# Autodesk Inventor assembly: Full-Assembly
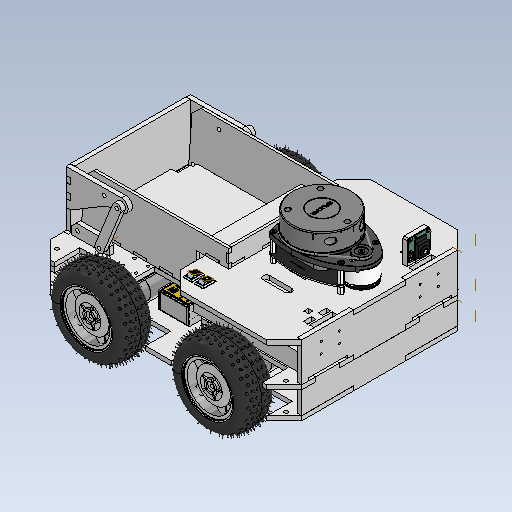
[picture p0: Inventor's stored thumbnail of the model, 512x512]
Saved by Autodesk Inventor 2025 (Build 290162000, 162)
## iProperties
Created: 2025-08-20
Part Number: Full-Assembly
Document SubType Name: Assembly
Designer: HP
Author: HP
## Documents named in this file (20)
- C:\Users\HP\Documents\GitHub\robotics-dojo-2025\CAD\Full-Assembly.iam
- C:\Users\HP\Documents\GitHub\robotics-dojo-2025\CAD\RP-lidar-A1\RP-lidar-A1.iam
- C:\Users\HP\Documents\GitHub\robotics-dojo-2025\CAD\lipo\TATTU 1800 3S.iam
- C:\Users\HP\Documents\GitHub\robotics-dojo-2025\CAD\wheel-assembly.iam
- C:\Users\HP\Documents\GitHub\robotics-dojo-2025\CAD\mainBoard.ipt
- C:\Users\HP\Documents\GitHub\robotics-dojo-2025\CAD\servo\MG-996R.ipt
- C:\Users\HP\Documents\GitHub\robotics-dojo-2025\CAD\pi\pi-assembly.iam
- C:\Users\HP\Documents\GitHub\robotics-dojo-2025\CAD\cam\raspicam_ai_assy.iam
- C:\Users\HP\Documents\GitHub\robotics-dojo-2025\CAD\frame.iam
- C:\Users\HP\Documents\GitHub\robotics-dojo-2025\CAD\servo-arm.ipt
- C:\Users\HP\Documents\GitHub\robotics-dojo-2025\CAD\lower-tipper-link.ipt
- C:\Users\HP\Documents\GitHub\robotics-dojo-2025\CAD\upper-tipper-link.ipt
- C:\Users\HP\Documents\GitHub\robotics-dojo-2025\CAD\gate.ipt
- C:\Users\HP\Documents\GitHub\robotics-dojo-2025\CAD\gate-anchor-link.ipt
- C:\Users\HP\Documents\GitHub\robotics-dojo-2025\CAD\gate-upper-link.ipt
- C:\Users\HP\Documents\GitHub\robotics-dojo-2025\CAD\power-bank.ipt
- C:\Users\HP\Documents\GitHub\robotics-dojo-2025\CAD\power-bank-bump.ipt
- C:\Users\HP\Documents\GitHub\robotics-dojo-2025\CAD\wheel\Off Road Tyre v3.ipt
- C:\Users\HP\Documents\GitHub\robotics-dojo-2025\CAD\bed_acrylic_assembly.iam
- C:\Users\HP\Documents\GitHub\robotics-dojo-2025\CAD\switch\power button.iam
## Components (29 placed, 19 different names)
1. RP-lidar-A1:1 [sub-assembly] — Insert:9, Insert:10
2. TATTU 1800 3S:1 [sub-assembly] — Mate:12, Flush:2, Mate:15
3. TATTU 1800 3S:2 [sub-assembly] — Mate:13, Flush:2, Mate:14, Mate:15, Mate:16
4. wheel-assembly:1 [sub-assembly] — Mate:4, Insert:3, Insert:4, Mate:57, Mate:58
5. wheel-assembly:2 [sub-assembly] — Mate:3, Insert:5, Insert:6, Mate:55, Mate:56
6. wheel-assembly:3 [sub-assembly] — Mate:1, Insert:1, Insert:2, Mate:16, Mate:51, Mate:52
7. wheel-assembly:4 [sub-assembly] — Mate:2, Insert:7, Insert:8, Mate:53, Mate:54
8. mainBoard:1 — Mate:5, Flush:7, Mate:23
9. MG-996R:1 — Mate:22, Insert:15, Flush:4, Flush:9
10. pi-assembly:1 [sub-assembly] — Mate:7, Flush:5, Flush:7, Mate:23, Mate:25
11. raspicam_ai_assy:1 [sub-assembly] — Mate:70, Mate:71, Mate:72
12. frame:1 [sub-assembly] — Mate:1, Mate:2, Mate:3, Mate:4, Insert:1, Insert:2, Insert:3, Insert:4, Insert:5, Insert:6, Insert:7, Insert:8, Mate:5, Mate:7, Mate:12, Mate:13, Mate:14, Insert:9, Insert:10, Mate:22, Flush:4, Flush:5, Mate:25, Flush:9, Insert:25, Insert:27, Mate:49, Mate:59, Mate:60, Flush:11, Mate:70, Mate:71, Mate:72, Mate:73, Mate:74, Mate:75, Mate:76, Mate:77, Mate:78, Angle:4
13. servo-arm:1 — Angle:1, Insert:15, Insert:18
14. lower-tipper-link:1 — Angle:1, Insert:18, Insert:19
15. upper-tipper-link:1 — Insert:19, Mate:61
16. gate:1 — Mate:38, Mate:39, Mate:40, Mate:42, Mate:43
17. gate-anchor-link:1 — Insert:25, Mate:44
18. gate-upper-link:1 — Mate:38, Mate:39, Mate:40, Mate:44, Mate:62
19. gate-upper-link:2 — Mate:42, Mate:43, Mate:46
20. gate-anchor-link:2 — Insert:27, Mate:46
21. power-bank:1 — Mate:49, Mate:50, Flush:10, Mate:59
22. power-bank-bump:1 — Mate:50, Flush:10
23. Off Road Tyre v3:1 — Mate:57, Mate:58, Angle:5
24. Off Road Tyre v3:2 — Mate:55, Mate:56, Angle:6
25. Off Road Tyre v3:3 — Mate:53, Mate:54, Angle:7
26. Off Road Tyre v3:4 — Mate:51, Mate:52, Angle:8
27. bed_acrylic_assembly:1 [sub-assembly] — Mate:60, Mate:61, Mate:62, Flush:11, Angle:4
28. power button:1 [sub-assembly] — Mate:74, Mate:75, Mate:78
29. power button:2 [sub-assembly] — Mate:73, Mate:76, Mate:77
## Relationships (72: Mate 44, Insert 15, Flush 7, Angle 6)
- Mate:1: wheel-assembly:3 ↔ frame:1
- Mate:2: wheel-assembly:4 ↔ frame:1
- Mate:3: wheel-assembly:2 ↔ frame:1
- Mate:4: wheel-assembly:1 ↔ frame:1
- Insert:1: wheel-assembly:3 ↔ frame:1
- Insert:2: wheel-assembly:3 ↔ frame:1
- Insert:3: wheel-assembly:1 ↔ frame:1
- Insert:4: wheel-assembly:1 ↔ frame:1
- Insert:5: wheel-assembly:2 ↔ frame:1
- Insert:6: wheel-assembly:2 ↔ frame:1
- Insert:7: wheel-assembly:4 ↔ frame:1
- Insert:8: wheel-assembly:4 ↔ frame:1
- Mate:5: mainBoard:1 ↔ frame:1
- Mate:7: pi-assembly:1 ↔ frame:1
- Mate:12: TATTU 1800 3S:1 ↔ frame:1
- Mate:13: TATTU 1800 3S:2 ↔ frame:1
- Flush:2: TATTU 1800 3S:1 ↔ TATTU 1800 3S:2
- Mate:14: TATTU 1800 3S:2 ↔ frame:1
- Insert:9: RP-lidar-A1:1 ↔ frame:1
- Insert:10: RP-lidar-A1:1 ↔ frame:1
- Mate:15 (15 mm): TATTU 1800 3S:1 ↔ TATTU 1800 3S:2
- Mate:16 (30 mm): TATTU 1800 3S:2 ↔ wheel-assembly:3
- Mate:22: MG-996R:1 ↔ frame:1
- Angle:1 (0 deg): servo-arm:1 ↔ lower-tipper-link:1
- Insert:15 (-4 mm): MG-996R:1 ↔ servo-arm:1
- Insert:18: servo-arm:1 ↔ lower-tipper-link:1
- Insert:19: lower-tipper-link:1 ↔ upper-tipper-link:1
- Flush:4: MG-996R:1 ↔ frame:1
- Flush:5: pi-assembly:1 ↔ frame:1
- Flush:7: mainBoard:1 ↔ pi-assembly:1
- Mate:23: mainBoard:1 ↔ pi-assembly:1
- Mate:25: pi-assembly:1 ↔ frame:1
- Flush:9: MG-996R:1 ↔ frame:1
- Insert:25: frame:1 ↔ gate-anchor-link:1
- Mate:38: gate:1 ↔ gate-upper-link:1
- Mate:39: gate:1 ↔ gate-upper-link:1
- Mate:40: gate:1 ↔ gate-upper-link:1
- Mate:42: gate:1 ↔ gate-upper-link:2
- Mate:43: gate:1 ↔ gate-upper-link:2
- Mate:44: gate-anchor-link:1 ↔ gate-upper-link:1
- Insert:27: frame:1 ↔ gate-anchor-link:2
- Mate:46: gate-upper-link:2 ↔ gate-anchor-link:2
- Mate:49: frame:1 ↔ power-bank:1
- Mate:50: power-bank:1 ↔ power-bank-bump:1
- Mate:51: wheel-assembly:3 ↔ Off Road Tyre v3:4
- Mate:52: wheel-assembly:3 ↔ Off Road Tyre v3:4
- Mate:53: wheel-assembly:4 ↔ Off Road Tyre v3:3
- Mate:54: wheel-assembly:4 ↔ Off Road Tyre v3:3
- Mate:55: wheel-assembly:2 ↔ Off Road Tyre v3:2
- Mate:56: wheel-assembly:2 ↔ Off Road Tyre v3:2
- Mate:57: wheel-assembly:1 ↔ Off Road Tyre v3:1
- Mate:58: wheel-assembly:1 ↔ Off Road Tyre v3:1
- Flush:10: power-bank:1 ↔ power-bank-bump:1
- Mate:59: frame:1 ↔ power-bank:1
- Mate:60: frame:1 ↔ bed_acrylic_assembly:1
- Mate:61: upper-tipper-link:1 ↔ bed_acrylic_assembly:1
- Mate:62: gate-upper-link:1 ↔ bed_acrylic_assembly:1
- Flush:11: frame:1 ↔ bed_acrylic_assembly:1
- Mate:70: raspicam_ai_assy:1 ↔ frame:1
- Mate:71: raspicam_ai_assy:1 ↔ frame:1
- Mate:72: raspicam_ai_assy:1 ↔ frame:1
- Mate:73: frame:1 ↔ power button:2
- Mate:74: frame:1 ↔ power button:1
- Mate:75: frame:1 ↔ power button:1
- Mate:76: frame:1 ↔ power button:2
- Mate:77: frame:1 ↔ power button:2
- Mate:78: frame:1 ↔ power button:1
- Angle:4 (0 deg): frame:1 ↔ bed_acrylic_assembly:1
- Angle:5 (0 deg): Off Road Tyre v3:1
- Angle:6 (0 deg): Off Road Tyre v3:2
- Angle:7 (0 deg): Off Road Tyre v3:3
- Angle:8 (0 deg): Off Road Tyre v3:4
